# Autodesk Inventor assembly: Bellows Assembly
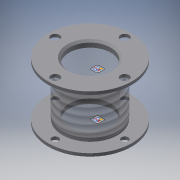
[picture p0: Inventor's stored thumbnail of the model, 180x180]
Saved by Autodesk Inventor 2019.4 (Build 234330000, 330)
## iProperties
Created: 2021-01-08
Part Number: Bellows Assembly
Document SubType Name: Assembly
Designer: caleb
Author: caleb
## Documents named in this file (4)
- C:\Users\cfang\Desktop\nebraska-silicon-lab\CAD\ETL\Module Assembly\Picker Tool\Bellows Assembly.iam
- C:\Users\cfang\Desktop\nebraska-silicon-lab\CAD\ETL\Module Assembly\Picker Tool\FC-13 Bellows.ipt
- C:\Users\cfang\Desktop\nebraska-silicon-lab\CAD\ETL\Module Assembly\Picker Tool\Flange_1.ipt
- C:\Users\cfang\Desktop\nebraska-silicon-lab\CAD\ETL\Module Assembly\Picker Tool\Flange_2.ipt
## Components (3 placed, 3 different names)
1. FC-13 Bellows:1 — Insert:1, Insert:2
2. Flange_1:1 — Insert:2
3. Flange_2:1 — Insert:1
## Relationships (2: Insert 2)
- Insert:1 (-1.1176 mm): FC-13 Bellows:1 ↔ Flange_2:1
- Insert:2 (-1.1176 mm): FC-13 Bellows:1 ↔ Flange_1:1
